# Autodesk Inventor assembly: daisen_motor
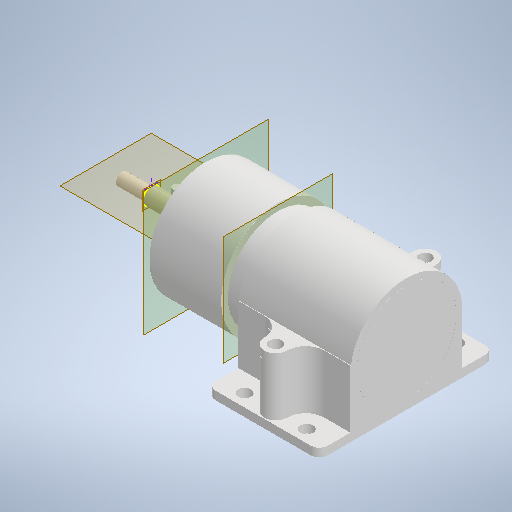
[picture p0: Inventor's stored thumbnail of the model, 512x512]
Saved by Autodesk Inventor 2025.2 (Build 292293000, 293)
## iProperties
Created: 2025-01-13
Part Number: daisen_motor
Document SubType Name: Assembly
Designer: mahhy
Author: mahhy
## Documents named in this file (5)
- D:\兵庫県立大\creap\daisen_motor\daisen_motor.iam
- D:\兵庫県立大\creap\daisen_motor\daisen_moto_parts1.ipt
- D:\兵庫県立大\creap\daisen_motor\daisen_moto_parts2.ipt
- D:\兵庫県立大\creap\daisen_motor\daisen_motor.ipt
- D:\兵庫県立大\creap\daisen_motor\daisen_motor_part3.ipt
## Components (4 placed, 4 different names)
1. daisen_moto_parts1:1 — リジッド:1
2. daisen_moto_parts2:1 — リジッド:1, 挿入:1
3. daisen_motor:1 — 挿入:1, リジッド:2
4. daisen_motor_part3:1 — リジッド:2
## Relationships (3: WeldJoint 2, Insert 1)
- リジッド:1 [WeldJoint]: daisen_moto_parts1:1 ↔ daisen_moto_parts2:1
- 挿入:1 [Insert]: daisen_moto_parts2:1 ↔ daisen_motor:1
- リジッド:2 [WeldJoint] (5 mm): daisen_motor:1 ↔ daisen_motor_part3:1
